# Autodesk Inventor assembly: Shaft Collar Metal
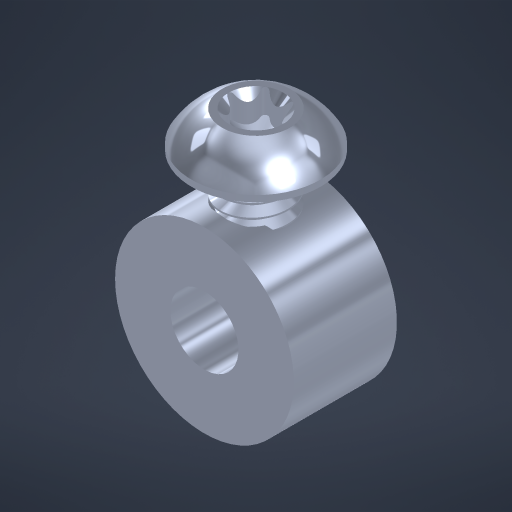
[picture p0: Inventor's stored thumbnail of the model, 512x512]
Saved by Autodesk Inventor 2023 (Build 270158000, 158)
## iProperties
Created: 2022-08-01
Part Number: Shaft Collar Metal
Document SubType Name: Assembly
Designer: ylu12
Author: ylu12
## Documents named in this file (5)
- C:\Users\eduar\VRC\CAD\Parts\standard\Motion\Shafts\Shaft Collar\Shaft Collar Star Threaded.iam
- C:\Users\eduar\VRC\CAD\Parts\standard\Motion\Shafts\Reference Parts\Shaft Collar Metal.ipt
- C:\Users\eduar\VRC\CAD\Parts\standard\Structure\Connectors\Screw Steel - Star\SScrew Star Threaded .250.ipt
- D:\CAD\Parts\standard\Structure\Connectors\Screw Steel - Star.ipt
- C:\Users\eduar\VRC\CAD\Parts\standard\Motion\Shafts\Shaft Collar.iam
## Components (2 placed, 2 different names)
1. Shaft Collar Metal:1 — Mate:1, Mate:2, Flush:1, Insert:3
2. SScrew Star Threaded .250:1 — Insert:3
## Relationships (4: Mate 2, Flush 1, Insert 1)
- Mate:1: Shaft Collar Metal:1
- Mate:2: Shaft Collar Metal:1
- Flush:1: Shaft Collar Metal:1
- Insert:3 (2.54 mm): Shaft Collar Metal:1 ↔ SScrew Star Threaded .250:1
